# Autodesk Inventor assembly: 3A.01.11.JS.Rib 11
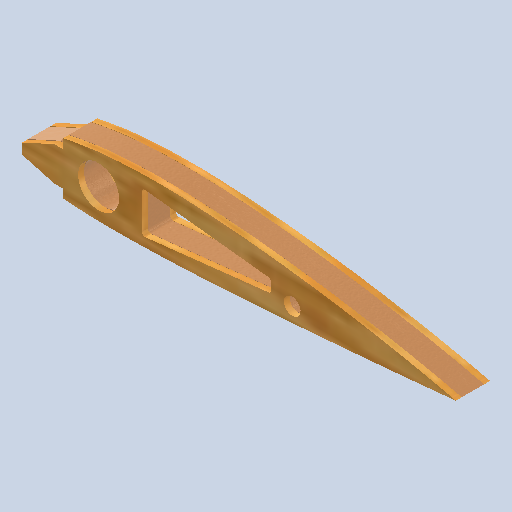
[picture p0: Inventor's stored thumbnail of the model, 512x512]
Saved by Autodesk Inventor 2025.1 (Build 291241000, 241)
## iProperties
Created: 2025-01-14
Part Number: 3A.01.11.JS.Rib 11
Document SubType Name: Assembly
Designer: johan
Author: johan
## Documents named in this file (3)
- C:\Users\johan\OneDrive - University of Bristol\CAD docs\2) Wing\2) Ribs\assemblies\3A.01.11.JS.Rib 11.iam
- C:\Users\johan\OneDrive - University of Bristol\CAD docs\2) Wing\2) Ribs\parts\Full length unmodified\3P.03.11.01.JS.rib 11 ply.ipt
- C:\Users\johan\OneDrive - University of Bristol\CAD docs\2) Wing\2) Ribs\parts\Full length unmodified\3P.03.11.02.JS.rib 11 foam.ipt
## Components (3 placed, 2 different names)
1. 3P.03.11.01.JS.rib 11 ply:1 — Rigid:2
2. 3P.03.11.02.JS.rib 11 foam:1 — Rigid:1, Rigid:2
3. 3P.03.11.01.JS.rib 11 ply:2 — Rigid:1
## Relationships (2: WeldJoint 2)
- Rigid:1 [WeldJoint]: 3P.03.11.02.JS.rib 11 foam:1 ↔ 3P.03.11.01.JS.rib 11 ply:2
- Rigid:2 [WeldJoint]: 3P.03.11.01.JS.rib 11 ply:1 ↔ 3P.03.11.02.JS.rib 11 foam:1
